# Autodesk Inventor assembly: FinalAssembly01
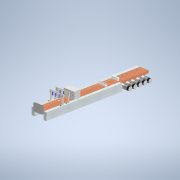
[picture p0: Inventor's stored thumbnail of the model, 180x180]
Saved by Autodesk Inventor 2021 (Build 250183000, 183)
## iProperties
Created: 2021-02-01
Part Number: FinalAssembly01
Document SubType Name: Assembly
Designer: garre
Author: garre
## Documents named in this file (14)
- C:\Users\Ryan\Documents\School\MQP\Case Model\Branch2\MQPInstrumentCAD-bodyModification\MQPInstrumentCAD-bodyModification\FinalAssembly01.iam
- C:\Users\Ryan\Documents\School\MQP\Case Model\Branch2\MQPInstrumentCAD-bodyModification\MQPInstrumentCAD-bodyModification\bodySidePlate.ipt
- C:\Users\Ryan\Documents\School\MQP\Case Model\Branch2\MQPInstrumentCAD-bodyModification\MQPInstrumentCAD-bodyModification\bodyTopPlate.ipt
- C:\Users\Ryan\Documents\School\MQP\Case Model\Branch2\MQPInstrumentCAD-bodyModification\MQPInstrumentCAD-bodyModification\bodyBotPlate.ipt
- C:\Users\Ryan\Documents\School\MQP\Case Model\Branch2\MQPInstrumentCAD-bodyModification\MQPInstrumentCAD-bodyModification\LoadCell.ipt
- C:\Users\Ryan\Documents\School\MQP\Case Model\Branch2\MQPInstrumentCAD-bodyModification\MQPInstrumentCAD-bodyModification\TuningPeg.ipt
- C:\Users\Ryan\Documents\School\MQP\Case Model\Branch2\MQPInstrumentCAD-bodyModification\MQPInstrumentCAD-bodyModification\MountedMotor.iam
- C:\Users\Ryan\Documents\School\MQP\Case Model\Branch2\MQPInstrumentCAD-bodyModification\MQPInstrumentCAD-bodyModification\bodySidePlateAlt.ipt
- C:\Users\Ryan\Documents\School\MQP\Case Model\Branch2\MQPInstrumentCAD-bodyModification\MQPInstrumentCAD-bodyModification\Nut0.ipt
- C:\Users\Ryan\Documents\School\MQP\Case Model\Branch2\MQPInstrumentCAD-bodyModification\MQPInstrumentCAD-bodyModification\String.ipt
- C:\Users\Ryan\Documents\School\MQP\Case Model\Branch2\MQPInstrumentCAD-bodyModification\MQPInstrumentCAD-bodyModification\PCB_Case.iam
- C:\Users\Ryan\Documents\School\MQP\Case Model\Branch2\MQPInstrumentCAD-bodyModification\MQPInstrumentCAD-bodyModification\Pickup.ipt
- C:\Users\Ryan\Documents\School\MQP\Case Model\Branch2\MQPInstrumentCAD-bodyModification\MQPInstrumentCAD-bodyModification\Frame.ipt
- C:\Users\Ryan\Documents\School\MQP\Case Model\Branch2\MQPInstrumentCAD-bodyModification\MQPInstrumentCAD-bodyModification\Solenoid.ipt
## Components (34 placed, 13 different names)
1. bodySidePlate:1 — Mate:2, Flush:3, Flush:4, Mate:4, Mate:10, Mate:25, Mate:52
2. bodyTopPlate:1 — Mate:2, Flush:3, Flush:4, Mate:5, Mate:6, Mate:7, Mate:8, Mate:9, Flush:6, Mate:37, Mate:38, Angle:1, Mate:39, Mate:54, Mate:55, Mate:56
3. bodySidePlateAlt:1 — Mate:37, Mate:38, Mate:51, Mate:53, Mate:57, Mate:58, Mate:59, Mate:60
4. PCB_Case:1 [sub-assembly] — Mate:51, Mate:52, Mate:53
5. Pickup:1 — Mate:54, Mate:55, Mate:56
6. MountedMotor:5 [sub-assembly] — Mate:34, Flush:20, Mate:35
7. MountedMotor:4 [sub-assembly] — Mate:32, Flush:19, Mate:33, Mate:35
8. MountedMotor:3 [sub-assembly] — Mate:30, Flush:18, Mate:31, Mate:33
9. MountedMotor:2 [sub-assembly] — Mate:28, Flush:17, Mate:29, Mate:31
10. MountedMotor:1 [sub-assembly] — Mate:26, Mate:27, Flush:16, Mate:29
11. TuningPeg:5 — Mate:15, Mate:21, Angle:4, Angle:5
12. TuningPeg:3 — Mate:16, Mate:19, Angle:2, Angle:3
13. TuningPeg:2 — Mate:14, Mate:20, Angle:3, Angle:4
14. TuningPeg:4 — Mate:17, Mate:22, Angle:5
15. TuningPeg:1 — Mate:13, Mate:18, Angle:1, Angle:2
16. bodyBotPlate:1 — Mate:4, Mate:13, Mate:14, Mate:15, Mate:16, Mate:17, Mate:18, Mate:19, Mate:20, Mate:21, Mate:22, Mate:25, Mate:26, Mate:27, Flush:16, Mate:28, Flush:17, Mate:30, Flush:18, Mate:32, Flush:19, Mate:34, Flush:20, Mate:40
17. String:5 — Mate:49, Mate:50
18. String:4 — Mate:47, Mate:48
19. String:3 — Mate:45, Mate:46
20. String:2 — Mate:43, Mate:44
21. String:1 — Mate:41, Mate:42
22. Nut0:1 — Mate:39, Mate:40, Mate:41, Mate:43, Mate:45, Mate:47, Mate:49
23. LoadCell:5 — Mate:9, Flush:9, Flush:14, Mate:10, Mate:50
24. LoadCell:4 — Mate:8, Flush:7, Flush:12, Flush:14, Mate:48
25. LoadCell:3 — Mate:7, Flush:8, Flush:13, Mate:42
26. LoadCell:2 — Mate:6, Flush:10, Flush:11, Flush:12, Mate:46
27. LoadCell:1 — Mate:5, Flush:6, Flush:7, Flush:8, Flush:9, Flush:10, Flush:11, Flush:13, Mate:44
28. Solenoid:5 — Mate:69, Mate:70
29. Solenoid:4 — Mate:67, Mate:68
30. Solenoid:3 — Mate:71, Mate:72
31. Solenoid:2 — Mate:63, Mate:64
32. Solenoid:1 — Mate:65, Mate:66
33. Frame:2 — Mate:60, Mate:61, Mate:62, Mate:67, Mate:68, Mate:69, Mate:70, Mate:71, Mate:72
34. Frame:1 — Mate:57, Mate:58, Mate:59, Mate:61, Mate:62, Mate:63, Mate:64, Mate:65, Mate:66
## Relationships (86: Mate 65, Flush 16, Angle 5)
- Mate:2: bodySidePlate:1 ↔ bodyTopPlate:1
- Flush:3: bodySidePlate:1 ↔ bodyTopPlate:1
- Flush:4: bodySidePlate:1 ↔ bodyTopPlate:1
- Mate:4: bodySidePlate:1 ↔ bodyBotPlate:1
- Mate:5: bodyTopPlate:1 ↔ LoadCell:1
- Mate:6: bodyTopPlate:1 ↔ LoadCell:2
- Mate:7: bodyTopPlate:1 ↔ LoadCell:3
- Mate:8: bodyTopPlate:1 ↔ LoadCell:4
- Mate:9: bodyTopPlate:1 ↔ LoadCell:5
- Flush:6: bodyTopPlate:1 ↔ LoadCell:1
- Flush:7: LoadCell:4 ↔ LoadCell:1
- Flush:8: LoadCell:3 ↔ LoadCell:1
- Flush:9: LoadCell:5 ↔ LoadCell:1
- Flush:10: LoadCell:2 ↔ LoadCell:1
- Flush:11 (15.875 mm): LoadCell:2 ↔ LoadCell:1
- Flush:12 (15.875 mm): LoadCell:4 ↔ LoadCell:2
- Flush:13 (15.875 mm): LoadCell:3 ↔ LoadCell:1
- Flush:14 (-15.875 mm): LoadCell:5 ↔ LoadCell:4
- Mate:10: bodySidePlate:1 ↔ LoadCell:5
- Mate:13: TuningPeg:1 ↔ bodyBotPlate:1
- Mate:14: TuningPeg:2 ↔ bodyBotPlate:1
- Mate:15: TuningPeg:5 ↔ bodyBotPlate:1
- Mate:16: TuningPeg:3 ↔ bodyBotPlate:1
- Mate:17: TuningPeg:4 ↔ bodyBotPlate:1
- Mate:18: TuningPeg:1 ↔ bodyBotPlate:1
- Mate:19: TuningPeg:3 ↔ bodyBotPlate:1
- Mate:20: TuningPeg:2 ↔ bodyBotPlate:1
- Mate:21: TuningPeg:5 ↔ bodyBotPlate:1
- Mate:22: TuningPeg:4 ↔ bodyBotPlate:1
- Mate:25: bodySidePlate:1 ↔ bodyBotPlate:1
- Mate:26: MountedMotor:1 ↔ bodyBotPlate:1
- Mate:27: MountedMotor:1 ↔ bodyBotPlate:1
- Flush:16 (36.83 mm): MountedMotor:1 ↔ bodyBotPlate:1
- Mate:28: MountedMotor:2 ↔ bodyBotPlate:1
- Flush:17: MountedMotor:2 ↔ bodyBotPlate:1
- Mate:29: MountedMotor:2 ↔ MountedMotor:1
- Mate:30: MountedMotor:3 ↔ bodyBotPlate:1
- Flush:18: MountedMotor:3 ↔ bodyBotPlate:1
- Mate:31: MountedMotor:3 ↔ MountedMotor:2
- Mate:32: MountedMotor:4 ↔ bodyBotPlate:1
- Flush:19: MountedMotor:4 ↔ bodyBotPlate:1
- Mate:33: MountedMotor:4 ↔ MountedMotor:3
- Mate:34: MountedMotor:5 ↔ bodyBotPlate:1
- Flush:20: MountedMotor:5 ↔ bodyBotPlate:1
- Mate:35: MountedMotor:5 ↔ MountedMotor:4
- Mate:37: bodyTopPlate:1 ↔ bodySidePlateAlt:1
- Mate:38: bodyTopPlate:1 ↔ bodySidePlateAlt:1
- Angle:1 (0 deg): bodyTopPlate:1 ↔ TuningPeg:1
- Angle:2 (0 deg): TuningPeg:3 ↔ TuningPeg:1
- Angle:3 (0 deg): TuningPeg:3 ↔ TuningPeg:2
- Angle:4 (0 deg): TuningPeg:5 ↔ TuningPeg:2
- Angle:5 (0 deg): TuningPeg:5 ↔ TuningPeg:4
- Mate:39: bodyTopPlate:1 ↔ Nut0:1
- Mate:40 (64.3509 mm): bodyBotPlate:1 ↔ Nut0:1
- Mate:41: String:1 ↔ Nut0:1
- Mate:42: String:1 ↔ LoadCell:3
- Mate:43: String:2 ↔ Nut0:1
- Mate:44: String:2 ↔ LoadCell:1
- Mate:45: String:3 ↔ Nut0:1
- Mate:46: String:3 ↔ LoadCell:2
- Mate:47: String:4 ↔ Nut0:1
- Mate:48: String:4 ↔ LoadCell:4
- Mate:49: String:5 ↔ Nut0:1
- Mate:50: String:5 ↔ LoadCell:5
- Mate:51: bodySidePlateAlt:1 ↔ PCB_Case:1
- Mate:52: bodySidePlate:1 ↔ PCB_Case:1
- Mate:53: bodySidePlateAlt:1 ↔ PCB_Case:1
- Mate:54: bodyTopPlate:1 ↔ Pickup:1
- Mate:55: bodyTopPlate:1 ↔ Pickup:1
- Mate:56: bodyTopPlate:1 ↔ Pickup:1
- Mate:57: bodySidePlateAlt:1 ↔ Frame:1
- Mate:58 (19.05 mm): bodySidePlateAlt:1 ↔ Frame:1
- Mate:59 (203.2 mm): bodySidePlateAlt:1 ↔ Frame:1
- Mate:60: bodySidePlateAlt:1 ↔ Frame:2
- Mate:61: Frame:2 ↔ Frame:1
- Mate:62 (76.2 mm): Frame:2 ↔ Frame:1
- Mate:63: Solenoid:2 ↔ Frame:1
- Mate:64 (77.978 mm): Solenoid:2 ↔ Frame:1
- Mate:65: Solenoid:1 ↔ Frame:1
- Mate:66 (63.754 mm): Solenoid:1 ↔ Frame:1
- Mate:67: Solenoid:4 ↔ Frame:2
- Mate:68 (21.844 mm): Solenoid:4 ↔ Frame:2
- Mate:69: Solenoid:5 ↔ Frame:2
- Mate:70 (64.008 mm): Solenoid:5 ↔ Frame:2
- Mate:71: Solenoid:3 ↔ Frame:2
- Mate:72 (35.814 mm): Solenoid:3 ↔ Frame:2
## Named parameters: loadCellWidth = 0 mm, stringSeparation = 12.7 mm, stringHorizontalOffset = 0 mm, loadCellSeparation = 3.175 mm, motorSeparation = 0 mm
